# Autodesk Inventor assembly: LEFT ARM
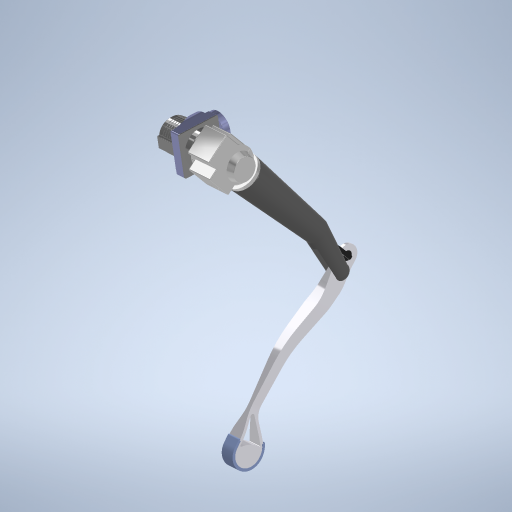
[picture p0: Inventor's stored thumbnail of the model, 512x512]
Saved by Autodesk Inventor 2023 (Build 270158000, 158)
## iProperties
Created: 2022-11-08
Part Number: LEFT ARM
Document SubType Name: Assembly
Designer: willy
Author: willy
## Documents named in this file (7)
- C:\Users\willy\Downloads\SPOT\LEFT ARM.iam
- C:\Users\willy\Downloads\SPOT\motor1_v2.ipt
- C:\Users\willy\Downloads\SPOT\motor2.ipt
- C:\Users\willy\Downloads\SPOT\motor3+fan.iam
- C:\Users\willy\Downloads\SPOT\spot_arm_v2.ipt
- C:\Users\willy\Downloads\SPOT\spot_foot.ipt
- C:\Users\willy\Downloads\SPOT\joint_v2.ipt
## Components (6 placed, 6 different names)
1. motor1_v2:1 — 삽입:1, 삽입:2, 삽입:3
2. motor2:1 — 삽입:1, 삽입:2
3. motor3+fan:1 [sub-assembly] — 삽입:3, 삽입:4, 삽입:5
4. spot_arm_v2:1 — 삽입:4, 삽입:5, 삽입:8, 메이트:3
5. spot_foot:1 — 메이트:1, 메이트:2, 삽입:7, 삽입:8
6. joint_v2:1 — 메이트:1, 메이트:2, 삽입:7, 메이트:3
## Relationships (10: Insert 7, Mate 3)
- 삽입:1 [Insert]: motor1_v2:1 ↔ motor2:1
- 삽입:2 [Insert]: motor1_v2:1 ↔ motor2:1
- 삽입:3 [Insert]: motor1_v2:1 ↔ motor3+fan:1
- 삽입:4 [Insert]: motor3+fan:1 ↔ spot_arm_v2:1
- 삽입:5 [Insert]: motor3+fan:1 ↔ spot_arm_v2:1
- 메이트:1 [Mate]: spot_foot:1 ↔ joint_v2:1
- 메이트:2 [Mate]: spot_foot:1 ↔ joint_v2:1
- 삽입:7 [Insert]: spot_foot:1 ↔ joint_v2:1
- 삽입:8 [Insert]: spot_arm_v2:1 ↔ spot_foot:1
- 메이트:3 [Mate]: spot_arm_v2:1 ↔ joint_v2:1
